# Autodesk Inventor assembly: collision3
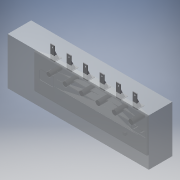
[picture p0: Inventor's stored thumbnail of the model, 180x180]
Saved by Autodesk Inventor 2018.1 (Build 221171000, 171)
## iProperties
Created: 2018-01-24
Part Number: collision3
Document SubType Name: Assembly
Designer: philippe
Author: philippe
## Documents named in this file (11)
- D:\EXCHANGE_MAINLINE2\prods\A3DPRCSDK\final-package\samples\exchange\exchangesource\Collision\data\ipt\collision3.iam
- D:\EXCHANGE_MAINLINE2\prods\A3DPRCSDK\final-package\samples\exchange\exchangesource\Collision\data\ipt\collision3_base.ipt
- D:\EXCHANGE_MAINLINE2\prods\A3DPRCSDK\final-package\samples\exchange\exchangesource\Collision\data\ipt\collision3_item.ipt
- D:\EXCHANGE_MAINLINE2\prods\A3DPRCSDK\final-package\samples\exchange\exchangesource\Collision\data\ipt\collision_cylinder_19_4.ipt
- D:\EXCHANGE_MAINLINE2\prods\A3DPRCSDK\final-package\samples\exchange\exchangesource\Collision\data\ipt\collision_cylinder_19_94.ipt
- D:\EXCHANGE_MAINLINE2\prods\A3DPRCSDK\final-package\samples\exchange\exchangesource\Collision\data\ipt\collision_cylinder_20.ipt
- D:\EXCHANGE_MAINLINE2\prods\A3DPRCSDK\final-package\samples\exchange\exchangesource\Collision\data\ipt\collision_cylinder_20_06.ipt
- D:\EXCHANGE_MAINLINE2\prods\A3DPRCSDK\final-package\samples\exchange\exchangesource\Collision\data\ipt\collision_cylinder_20_6.ipt
- D:\EXCHANGE_MAINLINE2\prods\A3DPRCSDK\final-package\samples\exchange\exchangesource\Collision\data\ipt\collision_cylinder_17_8.ipt
- D:\EXCHANGE_MAINLINE2\prods\A3DPRCSDK\final-package\samples\exchange\exchangesource\Collision\data\ipt\collision_big_box.ipt
- D:\EXCHANGE_MAINLINE2\prods\A3DPRCSDK\final-package\samples\exchange\exchangesource\Collision\data\ipt\collision_small_box.ipt
## Components (15 placed, 15 different names)
1. Base — Mate:1, Mate:2, Flush:1, Flush:2, Flush:3, Flush:4, Flush:5, Mate:3, Mate:4, Mate:5, Mate:6, Flush:6, Insert:1, Insert:2, Insert:4, Insert:5, Insert:6, Insert:7
2. Dist 0.0 — Mate:1, Flush:1, Flush:7
3. Dist -0.15 mm — Mate:6, Flush:6, Flush:7, Flush:8
4. Dist -0.03 mm — Flush:4, Mate:5, Flush:8, Flush:9
5. Dist 0.03 mm — Mate:2, Flush:2, Flush:9, Flush:10
6. Dist 0.3 mm — Flush:3, Mate:3, Flush:10, Flush:11
7. Dist 1.1mm — Flush:5, Mate:4, Flush:11
8. Cyl 0.0 mm — Insert:6
9. Cyl Dist -0.3mm — Insert:5
10. Cyl Dist -0.03mm — Insert:4
11. Cyl Dist 0.03mm — Insert:1
12. Cyl Dist 0.3 mm — Insert:2
13. Cyl Dist 1.1 mm — Insert:7
14. Big Box
15. Small Box
## Relationships (23: Flush 11, Mate 6, Insert 6)
- Mate:1: Base ↔ Dist 0.0
- Mate:2 (0.03 mm): Base ↔ Dist 0.03 mm
- Flush:1: Base ↔ Dist 0.0
- Flush:2: Base ↔ Dist 0.03 mm
- Flush:3: Base ↔ Dist 0.3 mm
- Flush:4: Base ↔ Dist -0.03 mm
- Flush:5: Base ↔ Dist 1.1mm
- Mate:3 (0.3 mm): Base ↔ Dist 0.3 mm
- Mate:4 (1.1 mm): Base ↔ Dist 1.1mm
- Mate:5 (-0.03 mm): Base ↔ Dist -0.03 mm
- Mate:6 (-0.15 mm): Base ↔ Dist -0.15 mm
- Flush:6: Base ↔ Dist -0.15 mm
- Flush:7 (70 mm): Dist 0.0 ↔ Dist -0.15 mm
- Flush:8 (70 mm): Dist -0.15 mm ↔ Dist -0.03 mm
- Flush:9 (70 mm): Dist -0.03 mm ↔ Dist 0.03 mm
- Flush:10 (70 mm): Dist 0.03 mm ↔ Dist 0.3 mm
- Flush:11 (70 mm): Dist 0.3 mm ↔ Dist 1.1mm
- Insert:1: Base ↔ Cyl Dist 0.03mm
- Insert:2: Base ↔ Cyl Dist 0.3 mm
- Insert:4: Base ↔ Cyl Dist -0.03mm
- Insert:5: Base ↔ Cyl Dist -0.3mm
- Insert:6: Base ↔ Cyl 0.0 mm
- Insert:7: Base ↔ Cyl Dist 1.1 mm
